# Autodesk Inventor assembly: !intake
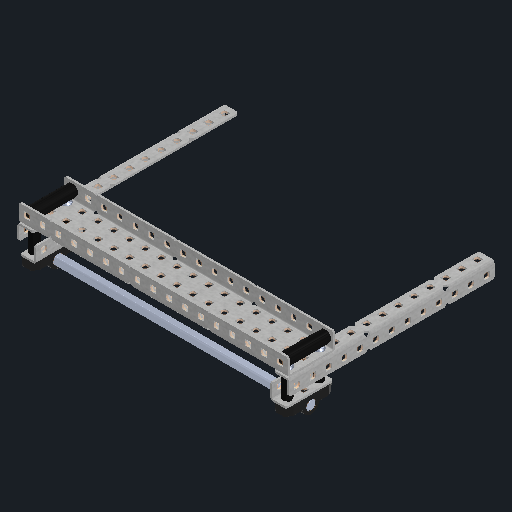
[picture p0: Inventor's stored thumbnail of the model, 512x512]
Saved by Autodesk Inventor 2025 (Build 290162000, 162)
## iProperties
Created: 2024-10-13
Part Number: !intake
Document SubType Name: Assembly
Designer: Averey Ku
Author: Averey Ku
## Documents named in this file (4)
- D:\vex_robotics_high_stakes\hardware\cad\bots\high_stakes_v2\intake\!intake.iam
- D:\vex_robotics_high_stakes\hardware\cad\bots\high_stakes_v2\intake\arm.iam
- D:\vex_robotics_high_stakes\hardware\cad\robpros_cad_lib\Motion\Shaft HS\Shaft HS\Shaft HS 8.5 in.ipt
- D:\vex_robotics_high_stakes\hardware\cad\robpros_cad_lib\Motion\Shaft HS\Shaft HS.ipt
## Components (2 placed, 2 different names)
1. arm:1 [sub-assembly] — Insert:1
2. Shaft HS 8.5 in:1 — Insert:1
## Relationships (1: Insert 1)
- Insert:1: arm:1 ↔ Shaft HS 8.5 in:1
